# Autodesk Inventor assembly: катушка+мотор
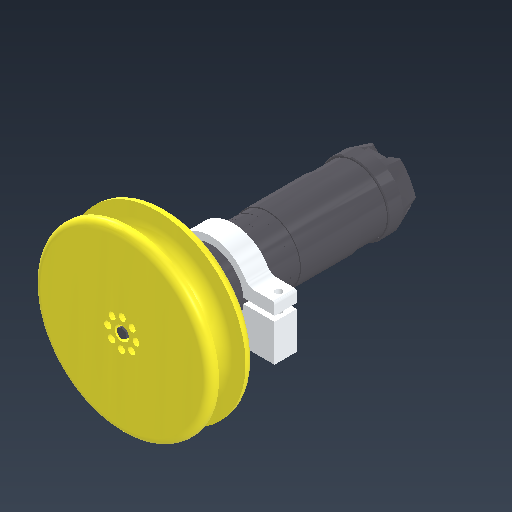
[picture p0: Inventor's stored thumbnail of the model, 512x512]
Saved by Autodesk Inventor 2025 (Build 290162000, 162)
## iProperties
Created: 2025-01-28
Part Number: катушка+мотор
Document SubType Name: Assembly
Designer: GameHD
Author: GameHD
## Documents named in this file (5)
- C:\Users\GameHD\Desktop\phantom 16950\катушка+мотор.iam
- C:\Users\GameHD\Desktop\phantom 16950\katushechka_pushechka\katushechka_pushechka.ipt
- C:\Users\GameHD\Desktop\phantom 16950\katushechka_pushechka 2\katushechka_pushechka 2.ipt
- C:\Users\GameHD\Desktop\phantom 16950\39089_txm-motormount\39089_txm-motormount.ipt
- C:\Users\GameHD\Desktop\phantom 16950\REV-41-1211\REV-41-1211.ipt
## Components (4 placed, 4 different names)
1. katushechka_pushechka:1
2. katushechka_pushechka 2:1
3. 39089_txm-motormount:1
4. REV-41-1211:1
## Relationships (5: Mate 4, Flush 1)
- [Mate]: katushechka_pushechka:1 ↔ katushechka_pushechka 2:1
- [Mate]: katushechka_pushechka:1 ↔ katushechka_pushechka 2:1
- [Mate]: 39089_txm-motormount:1 ↔ REV-41-1211:1
- [Mate]: katushechka_pushechka 2:1 ↔ REV-41-1211:1
- [Flush]: katushechka_pushechka 2:1 ↔ REV-41-1211:1
